# Autodesk Inventor assembly: PIVOT
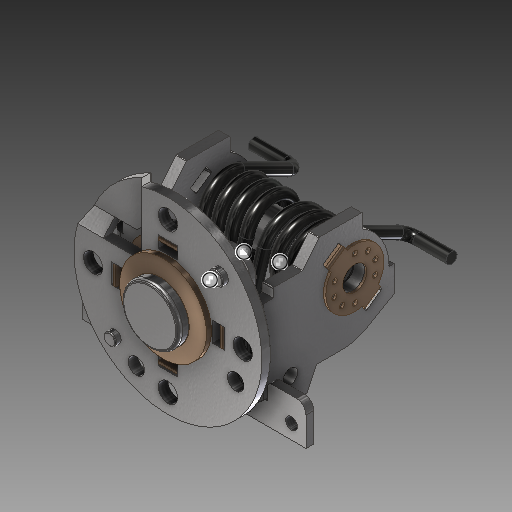
[picture p0: Inventor's stored thumbnail of the model, 512x512]
Saved by Autodesk Inventor 2017 SP1 (Build 210196100, 196)
## iProperties
Created: 2021-01-31
Part Number: PIVOT
Document SubType Name: Assembly
Designer: Napoleon
Author: Napoleon
## Documents named in this file (6)
- D:\PRYWATNE\PROJEKTY\POKÓJ\URZĄDZENIA PERYFERYJNE\DELL 1909Wf\PIVOT.iam
- D:\PRYWATNE\PROJEKTY\POKÓJ\URZĄDZENIA PERYFERYJNE\DELL 1909Wf\BLOKADA.iam
- D:\PRYWATNE\PROJEKTY\POKÓJ\URZĄDZENIA PERYFERYJNE\DELL 1909Wf\PODKŁADKA M8X6X18.ipt
- C:\Users\Administrator\Documents\Inventor\Content Center Files\R2017\pl-PL\ANSI B18.16.3M(2)\ANSI B18.16.3M - Property Class 5 and 10 - Metric M6 x 1 Typ metalowy.ipt
- D:\PRYWATNE\PROJEKTY\POKÓJ\URZĄDZENIA PERYFERYJNE\DELL 1909Wf\KOSZYK + ŁĄCZNIK.iam
- D:\PRYWATNE\PROJEKTY\POKÓJ\URZĄDZENIA PERYFERYJNE\DELL 1909Wf\Zespół1.iam
## Components (5 placed, 5 different names)
1. BLOKADA:2 [sub-assembly] — Sztywne:1, Obrotowe:1
2. PODKŁADKA M8X6X18:1 — Sztywne:1, Wstaw:1
3. KOSZYK + ŁĄCZNIK:1 [sub-assembly] — Obrotowe:1, Walcowe:1
4. Nakrętka samozabezpieczająca - Stal Metryczny Property Class 5 and 10 - Metric M6 x 1 Typ metalowy:2 — Wstaw:1
5. Zespół1:1 [sub-assembly] — Walcowe:1
## Relationships (4: WeldJoint 1, RevoluteJoint 1, Insert 1, CylindricalJoint 1)
- Sztywne:1 [WeldJoint] (-7.187 mm): BLOKADA:2 ↔ PODKŁADKA M8X6X18:1
- Obrotowe:1 [RevoluteJoint]: BLOKADA:2 ↔ KOSZYK + ŁĄCZNIK:1
- Wstaw:1 [Insert]: PODKŁADKA M8X6X18:1 ↔ Nakrętka samozabezpieczająca - Stal Metryczny Property Class 5 and 10 - Metric M6 x 1 Typ metalowy:2
- Walcowe:1 [CylindricalJoint]: KOSZYK + ŁĄCZNIK:1 ↔ Zespół1:1
